# Autodesk Inventor assembly: base_left
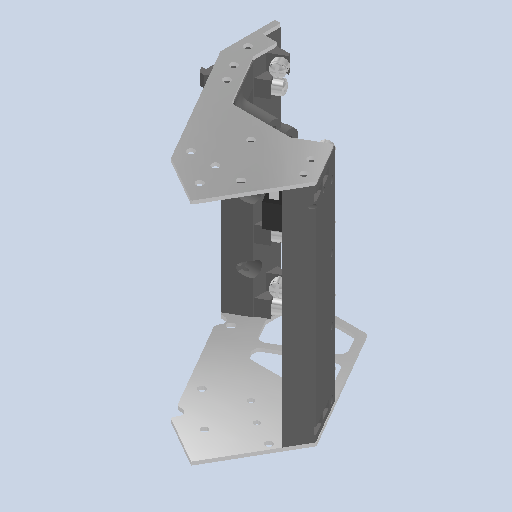
[picture p0: Inventor's stored thumbnail of the model, 512x512]
Saved by Autodesk Inventor 2024.1 (Build 281209000, 209)
## iProperties
Created: 2025-01-17
Part Number: base_left
Document SubType Name: Assembly
Designer: hibik
Author: hibik
## Documents named in this file (7)
- C:\Users\hibik\Documents\Robomech\RESCUE\ORCA\hard\fork\left\base_left.iam
- C:\Users\hibik\Documents\Robomech\RESCUE\ORCA\hard\fork\left\base_base_left.ipt
- C:\Users\hibik\Documents\Robomech\RESCUE\ORCA\hard\fork\left\bearing_3_6_2.5_left.ipt
- C:\Users\hibik\Documents\Robomech\RESCUE\ORCA\hard\fork\left\base_bearingpole_side_left.ipt
- C:\Users\hibik\Documents\Robomech\RESCUE\ORCA\hard\fork\left\base_cover_left.ipt
- C:\Users\hibik\Documents\Robomech\RESCUE\ORCA\hard\fork\left\limit_switch_left.ipt
- C:\Users\hibik\Documents\Robomech\RESCUE\ORCA\hard\fork\left\base_bearingpole_front_assy_left.iam
## Components (21 placed, 6 different names)
1. base_base_left:1 — フラッシュ:4, フラッシュ:3, メイト:2, フラッシュ:6, フラッシュ:5, 挿入:21
2. bearing_3_6_2.5_left:1 — 挿入:31
3. bearing_3_6_2.5_left:2 — 挿入:30
4. bearing_3_6_2.5_left:3 — 挿入:29
5. bearing_3_6_2.5_left:4 — 挿入:28
6. bearing_3_6_2.5_left:5 — 挿入:27
7. bearing_3_6_2.5_left:6 — 挿入:26
8. bearing_3_6_2.5_left:7 — 挿入:24
9. bearing_3_6_2.5_left:8 — 挿入:25
10. base_bearingpole_side_left:1 — フラッシュ:4, フラッシュ:3, メイト:2, 挿入:9, 挿入:10, 挿入:11, 挿入:12, 挿入:13, 挿入:14, 挿入:15, 挿入:16, メイト:3, 挿入:20, 挿入:19
11. bearing_3_6_2.5_left:9 — 挿入:9
12. bearing_3_6_2.5_left:10 — 挿入:10
13. bearing_3_6_2.5_left:11 — 挿入:11
14. bearing_3_6_2.5_left:12 — 挿入:12
15. bearing_3_6_2.5_left:13 — 挿入:13
16. bearing_3_6_2.5_left:14 — 挿入:14
17. bearing_3_6_2.5_left:15 — 挿入:15
18. bearing_3_6_2.5_left:16 — 挿入:16
19. base_cover_left:1 — フラッシュ:6, フラッシュ:5, メイト:3, 挿入:23, 挿入:22
20. limit_switch_left:2 — 挿入:20, 挿入:19
21. base_bearingpole_front_assy_left:1 [sub-assembly] — 挿入:31, 挿入:30, 挿入:29, 挿入:28, 挿入:27, 挿入:26, 挿入:25, 挿入:24, 挿入:23, 挿入:22, 挿入:21
## Relationships (27: Insert 21, Flush 4, Mate 2)
- フラッシュ:4 [Flush]: base_base_left:1 ↔ base_bearingpole_side_left:1
- フラッシュ:3 [Flush]: base_base_left:1 ↔ base_bearingpole_side_left:1
- メイト:2 [Mate]: base_base_left:1 ↔ base_bearingpole_side_left:1
- 挿入:9 [Insert]: base_bearingpole_side_left:1 ↔ bearing_3_6_2.5_left:9
- 挿入:10 [Insert]: base_bearingpole_side_left:1 ↔ bearing_3_6_2.5_left:10
- 挿入:11 [Insert]: base_bearingpole_side_left:1 ↔ bearing_3_6_2.5_left:11
- 挿入:12 [Insert]: base_bearingpole_side_left:1 ↔ bearing_3_6_2.5_left:12
- 挿入:13 [Insert]: base_bearingpole_side_left:1 ↔ bearing_3_6_2.5_left:13
- 挿入:14 [Insert]: base_bearingpole_side_left:1 ↔ bearing_3_6_2.5_left:14
- 挿入:15 [Insert]: base_bearingpole_side_left:1 ↔ bearing_3_6_2.5_left:15
- 挿入:16 [Insert]: base_bearingpole_side_left:1 ↔ bearing_3_6_2.5_left:16
- フラッシュ:6 [Flush]: base_base_left:1 ↔ base_cover_left:1
- フラッシュ:5 [Flush]: base_base_left:1 ↔ base_cover_left:1
- メイト:3 [Mate]: base_bearingpole_side_left:1 ↔ base_cover_left:1
- 挿入:20 [Insert]: base_bearingpole_side_left:1 ↔ limit_switch_left:2
- 挿入:19 [Insert]: base_bearingpole_side_left:1 ↔ limit_switch_left:2
- 挿入:31 [Insert]: bearing_3_6_2.5_left:1 ↔ base_bearingpole_front_assy_left:1
- 挿入:30 [Insert]: bearing_3_6_2.5_left:2 ↔ base_bearingpole_front_assy_left:1
- 挿入:29 [Insert]: bearing_3_6_2.5_left:3 ↔ base_bearingpole_front_assy_left:1
- 挿入:28 [Insert]: bearing_3_6_2.5_left:4 ↔ base_bearingpole_front_assy_left:1
- 挿入:27 [Insert]: bearing_3_6_2.5_left:5 ↔ base_bearingpole_front_assy_left:1
- 挿入:26 [Insert]: bearing_3_6_2.5_left:6 ↔ base_bearingpole_front_assy_left:1
- 挿入:25 [Insert]: bearing_3_6_2.5_left:8 ↔ base_bearingpole_front_assy_left:1
- 挿入:24 [Insert]: bearing_3_6_2.5_left:7 ↔ base_bearingpole_front_assy_left:1
- 挿入:23 [Insert]: base_cover_left:1 ↔ base_bearingpole_front_assy_left:1
- 挿入:22 [Insert]: base_cover_left:1 ↔ base_bearingpole_front_assy_left:1
- 挿入:21 [Insert]: base_base_left:1 ↔ base_bearingpole_front_assy_left:1
